# Autodesk Inventor assembly: Battery Pack - Samsung 25R
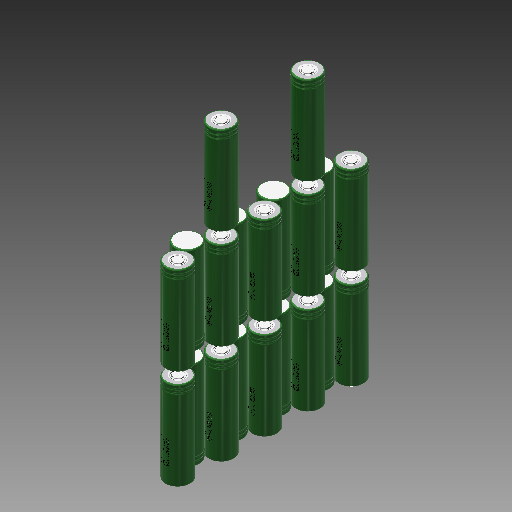
[picture p0: Inventor's stored thumbnail of the model, 512x512]
Saved by Autodesk Inventor 2019.3 (Build 233278000, 278)
## iProperties
Created: 2019-03-02
Part Number: Battery Pack - Samsung 25R
Document SubType Name: Assembly
Designer: Petar
Mass: 3015.47 g
Surface Area: 846.705 cm^2
Volume: 341.503 cm^3
Density: 8.83 g/cm^3
Author: Petar
## Documents named in this file (2)
- D:\OMG\E-Board\CAD\Inventor\Electrical Components\Battery Pack\Samsung 25R\Battery Pack - Samsung 25R -120deg.iam
- D:\OMG\E-Board\CAD\Inventor\Electrical Components\Battery Cell - Samsung.ipt
## Components (20 placed, 1 different names)
1. Battery Cell - Samsung:1 — Flush:1, Tangent:1, Angle:1, Mate:1, Flush:5, Flush:6, Mate:10, Mate:11
2. Battery Cell - Samsung:2 — Flush:1, Tangent:1, Angle:1, Mate:1, Tangent:4
3. Battery Cell - Samsung:3 — Flush:5, Tangent:4, Flush:6, Flush:11, Flush:12
4. Battery Cell - Samsung:4 — Tangent:8
5. Battery Cell - Samsung:5 — Flush:11, Flush:12, Tangent:8, Flush:16, Flush:17, Mate:13
6. Battery Cell - Samsung:6 — Tangent:11
7. Battery Cell - Samsung:7 — Flush:16, Tangent:11, Flush:17
8. Battery Cell - Samsung:8
9. Battery Cell - Samsung:9 — Mate:12
10. Battery Cell - Samsung:10 — Mate:10, Mate:11
11. Battery Cell - Samsung:11
12. Battery Cell - Samsung:12 — Mate:14, Mate:15
13. Battery Cell - Samsung:13
14. Battery Cell - Samsung:14 — Mate:13
15. Battery Cell - Samsung:15
16. Battery Cell - Samsung:16 — Mate:16, Mate:17
17. Battery Cell - Samsung:17
18. Battery Cell - Samsung:18 — Mate:12
19. Battery Cell - Samsung:19 — Mate:14, Mate:15
20. Battery Cell - Samsung:20 — Mate:16, Mate:17
## Relationships (64: Flush 24, Tangent 16, Mate 16, Angle 8)
- Flush:1: Battery Cell - Samsung:1 ↔ Battery Cell - Samsung:2
- Tangent:1: Battery Cell - Samsung:1 ↔ Battery Cell - Samsung:2
- Angle:1 (120 deg): Battery Cell - Samsung:1 ↔ Battery Cell - Samsung:2
- Mate:1 (-9.156 mm): Battery Cell - Samsung:1 ↔ Battery Cell - Samsung:2
- [Flush]: Battery Cell - Samsung:3 ↔ Battery Cell - Samsung:4
- [Tangent]: Battery Cell - Samsung:3 ↔ Battery Cell - Samsung:4
- [Angle] (120 deg): Battery Cell - Samsung:3 ↔ Battery Cell - Samsung:4
- [Mate] (-9.156 mm): Battery Cell - Samsung:3 ↔ Battery Cell - Samsung:4
- Flush:5: Battery Cell - Samsung:1 ↔ Battery Cell - Samsung:3
- Tangent:4: Battery Cell - Samsung:2 ↔ Battery Cell - Samsung:3
- Flush:6: Battery Cell - Samsung:1 ↔ Battery Cell - Samsung:3
- [Flush]: Battery Cell - Samsung:5 ↔ Battery Cell - Samsung:6
- [Tangent]: Battery Cell - Samsung:5 ↔ Battery Cell - Samsung:6
- [Angle] (120 deg): Battery Cell - Samsung:5 ↔ Battery Cell - Samsung:6
- [Mate] (-9.156 mm): Battery Cell - Samsung:5 ↔ Battery Cell - Samsung:6
- Flush:11: Battery Cell - Samsung:3 ↔ Battery Cell - Samsung:5
- Flush:12: Battery Cell - Samsung:3 ↔ Battery Cell - Samsung:5
- Tangent:8: Battery Cell - Samsung:4 ↔ Battery Cell - Samsung:5
- [Flush]: Battery Cell - Samsung:7 ↔ Battery Cell - Samsung:8
- [Tangent]: Battery Cell - Samsung:7 ↔ Battery Cell - Samsung:8
- [Angle] (120 deg): Battery Cell - Samsung:7 ↔ Battery Cell - Samsung:8
- [Mate] (-9.156 mm): Battery Cell - Samsung:7 ↔ Battery Cell - Samsung:8
- [Flush]: Battery Cell - Samsung:7 ↔ Battery Cell - Samsung:9
- [Tangent]: Battery Cell - Samsung:8 ↔ Battery Cell - Samsung:9
- [Flush]: Battery Cell - Samsung:7 ↔ Battery Cell - Samsung:9
- Flush:16: Battery Cell - Samsung:5 ↔ Battery Cell - Samsung:7
- Tangent:11: Battery Cell - Samsung:6 ↔ Battery Cell - Samsung:7
- Flush:17: Battery Cell - Samsung:5 ↔ Battery Cell - Samsung:7
- [Flush]: Battery Cell - Samsung:10 ↔ Battery Cell - Samsung:11
- [Tangent]: Battery Cell - Samsung:10 ↔ Battery Cell - Samsung:11
- [Angle] (120 deg): Battery Cell - Samsung:10 ↔ Battery Cell - Samsung:11
- [Mate] (-9.156 mm): Battery Cell - Samsung:10 ↔ Battery Cell - Samsung:11
- [Flush]: Battery Cell - Samsung:12 ↔ Battery Cell - Samsung:13
- [Tangent]: Battery Cell - Samsung:12 ↔ Battery Cell - Samsung:13
- [Angle] (120 deg): Battery Cell - Samsung:12 ↔ Battery Cell - Samsung:13
- [Mate] (-9.156 mm): Battery Cell - Samsung:12 ↔ Battery Cell - Samsung:13
- [Flush]: Battery Cell - Samsung:10 ↔ Battery Cell - Samsung:12
- [Tangent]: Battery Cell - Samsung:11 ↔ Battery Cell - Samsung:12
- [Flush]: Battery Cell - Samsung:10 ↔ Battery Cell - Samsung:12
- [Flush]: Battery Cell - Samsung:14 ↔ Battery Cell - Samsung:15
- [Tangent]: Battery Cell - Samsung:14 ↔ Battery Cell - Samsung:15
- [Angle] (120 deg): Battery Cell - Samsung:14 ↔ Battery Cell - Samsung:15
- [Mate] (-9.156 mm): Battery Cell - Samsung:14 ↔ Battery Cell - Samsung:15
- [Flush]: Battery Cell - Samsung:12 ↔ Battery Cell - Samsung:14
- [Flush]: Battery Cell - Samsung:12 ↔ Battery Cell - Samsung:14
- [Tangent]: Battery Cell - Samsung:13 ↔ Battery Cell - Samsung:14
- [Flush]: Battery Cell - Samsung:16 ↔ Battery Cell - Samsung:17
- [Tangent]: Battery Cell - Samsung:16 ↔ Battery Cell - Samsung:17
- [Angle] (120 deg): Battery Cell - Samsung:16 ↔ Battery Cell - Samsung:17
- [Mate] (-9.156 mm): Battery Cell - Samsung:16 ↔ Battery Cell - Samsung:17
- [Flush]: Battery Cell - Samsung:16 ↔ Battery Cell - Samsung:18
- [Tangent]: Battery Cell - Samsung:17 ↔ Battery Cell - Samsung:18
- [Flush]: Battery Cell - Samsung:16 ↔ Battery Cell - Samsung:18
- [Flush]: Battery Cell - Samsung:14 ↔ Battery Cell - Samsung:16
- [Tangent]: Battery Cell - Samsung:15 ↔ Battery Cell - Samsung:16
- [Flush]: Battery Cell - Samsung:14 ↔ Battery Cell - Samsung:16
- Mate:10 (8 mm): Battery Cell - Samsung:1 ↔ Battery Cell - Samsung:10
- Mate:11: Battery Cell - Samsung:1 ↔ Battery Cell - Samsung:10
- Mate:12: Battery Cell - Samsung:9 ↔ Battery Cell - Samsung:18
- Mate:13: Battery Cell - Samsung:5 ↔ Battery Cell - Samsung:14
- Mate:14 (8 mm): Battery Cell - Samsung:12 ↔ Battery Cell - Samsung:19
- Mate:15: Battery Cell - Samsung:12 ↔ Battery Cell - Samsung:19
- Mate:16 (8 mm): Battery Cell - Samsung:16 ↔ Battery Cell - Samsung:20
- Mate:17: Battery Cell - Samsung:16 ↔ Battery Cell - Samsung:20
## Named parameters: d65_d58 = 0 mm, d66_d59 = 0 mm, d67_d60 = 120 deg, d68_d64 = -9.156 mm, d75_d58 = 0 mm, d76_d59 = 0 mm, d77_d60 = 120 deg, d78_d64 = -9.156 mm, d86_d69 = 0 mm, d87_d70 = 0 mm, d88_d71 = 0 mm, d89_d58 = 0 mm, d90_d59 = 0 mm, d91_d60 = 120 deg, d92_d64 = -9.156 mm, d169_d168 = 0 mm, d170_d93 = 0 mm, d171_d95 = 0 mm, d172_d69 = 0 mm, d173_d70 = 0 mm, d174_d71 = 0 mm, d175_d75_d58 = 0 mm, d176_d76_d59 = 0 mm, d177_d77_d60 = 120 deg, d178_d78_d64 = -9.156 mm, d179_d83 = 0 mm, d180_d84 = 0 mm, d181_d85 = 0 mm, d182_d86_d69 = 0 mm, d183_d87_d70 = 0 mm, d184_d88_d71 = 0 mm, d185_d89_d58 = 0 mm, d186_d90_d59 = 0 mm, d187_d91_d60 = 120 deg, d188_d92_d64 = -9.156 mm, d189_d58 = 0 mm, d190_d59 = 0 mm, d191_d60 = 120 deg, d192_d64 = -9.156 mm, d193_d65_d58 = 0 mm, d194_d66_d59 = 0 mm, d195_d67_d60 = 120 deg, d196_d68_d64 = -9.156 mm
